# Autodesk Inventor assembly: Ensamblaje
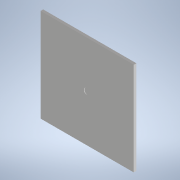
[picture p0: Inventor's stored thumbnail of the model, 180x180]
Saved by Autodesk Inventor 2020 (Build 240168000, 168)
## iProperties
Created: 2019-09-28
Part Number: Ensamblaje
Document SubType Name: Assembly
Designer: Java9
Author: Java9
## Documents named in this file (3)
- C:\Users\Java9\OneDrive\Documentos\Universidad\7mo\Cinemática de Robots\Nueva carpeta\Ensamblaje.iam
- C:\Users\Java9\OneDrive\Documentos\Universidad\7mo\Cinemática de Robots\Nueva carpeta\Base.ipt
- C:\Users\Java9\OneDrive\Documentos\Universidad\7mo\Cinemática de Robots\Nueva carpeta\plato.ipt
## Components (2 placed, 2 different names)
1. Base:1 — De rotación:1
2. plato:1 — De rotación:1
## Relationships (1: RevoluteJoint 1)
- De rotación:1 [RevoluteJoint]: Base:1 ↔ plato:1
